# Autodesk Inventor assembly: X_Carriage_V2_1
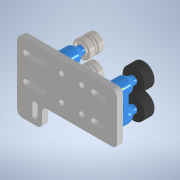
[picture p0: Inventor's stored thumbnail of the model, 180x180]
Saved by Autodesk Inventor 2021 (Build 250183000, 183)
## iProperties
Created: 2021-06-13
Part Number: X_Carriage_V2_1
Document SubType Name: Assembly
Designer: Jorian Brusind
Author: Jorian Brusind
## Documents named in this file (6)
- C:\Users\Jorian Brusind\Documents\GitHub\PersonalProjects\HyperRail\Inventor Files\X_Carriage_V2_1.iam
- C:\Users\Jorian Brusind\Documents\GitHub\PersonalProjects\HyperRail\Inventor Files\X_Carriage_Plate.ipt
- C:\Users\Jorian Brusind\Documents\GitHub\PersonalProjects\HyperRail\Inventor Files\11mm_BearingWheel.ipt
- C:\Users\Jorian Brusind\Documents\GitHub\PersonalProjects\HyperRail\Inventor Files\4mm_Roller_Spacer_extended.ipt
- C:\Users\Jorian Brusind\Documents\GitHub\PersonalProjects\HyperRail\Inventor Files\606zz_bearing.ipt
- C:\Users\Jorian Brusind\Documents\GitHub\PersonalProjects\HyperRail\Inventor Files\Bearing_Spacer.ipt
## Components (11 placed, 5 different names)
1. X_Carriage_Plate:1 — Mate:51, Mate:53, Mate:65, Angle:1, Mate:66, Angle:2
2. 11mm_BearingWheel:1 — Flush:2, Mate:56, Mate:67
3. 11mm_BearingWheel:4 — Flush:2, Mate:57
4. 4mm_Roller_Spacer_extended:1 — Mate:53, Mate:56, Mate:57, Mate:66, Angle:2, Mate:67
5. 4mm_Roller_Spacer_extended:2 — Mate:51, Mate:62, Mate:63, Mate:64, Mate:65, Angle:1
6. 606zz_bearing:1 — Mate:68, Mate:72
7. 606zz_bearing:2 — Mate:63, Mate:71
8. 606zz_bearing:3 — Mate:64, Mate:69
9. 606zz_bearing:4 — Mate:62, Mate:70
10. Bearing_Spacer:1 — Mate:69, Mate:70, Flush:4
11. Bearing_Spacer:2 — Mate:68, Mate:71, Flush:4, Mate:72
## Relationships (22: Mate 17, Flush 3, Angle 2)
- Flush:2: 11mm_BearingWheel:1 ↔ 11mm_BearingWheel:4
- Mate:51: X_Carriage_Plate:1 ↔ 4mm_Roller_Spacer_extended:2
- Mate:53: X_Carriage_Plate:1 ↔ 4mm_Roller_Spacer_extended:1
- Mate:56: 11mm_BearingWheel:1 ↔ 4mm_Roller_Spacer_extended:1
- Mate:57: 11mm_BearingWheel:4 ↔ 4mm_Roller_Spacer_extended:1
- [Mate]: 606zz_bearing:1 ↔ 606zz_bearing:2
- [Mate]: 606zz_bearing:3 ↔ 606zz_bearing:4
- [Flush]: 606zz_bearing:1 ↔ 606zz_bearing:3
- Mate:62: 4mm_Roller_Spacer_extended:2 ↔ 606zz_bearing:4
- Mate:63: 4mm_Roller_Spacer_extended:2 ↔ 606zz_bearing:2
- Mate:64: 4mm_Roller_Spacer_extended:2 ↔ 606zz_bearing:3
- Mate:65 (-12.5 mm): X_Carriage_Plate:1 ↔ 4mm_Roller_Spacer_extended:2
- Angle:1 (0 deg): X_Carriage_Plate:1 ↔ 4mm_Roller_Spacer_extended:2
- Mate:66 (-12.5 mm): X_Carriage_Plate:1 ↔ 4mm_Roller_Spacer_extended:1
- Angle:2 (0 deg): X_Carriage_Plate:1 ↔ 4mm_Roller_Spacer_extended:1
- Mate:67: 11mm_BearingWheel:1 ↔ 4mm_Roller_Spacer_extended:1
- Mate:68: 606zz_bearing:1 ↔ Bearing_Spacer:2
- Mate:69: 606zz_bearing:3 ↔ Bearing_Spacer:1
- Mate:70: 606zz_bearing:4 ↔ Bearing_Spacer:1
- Mate:71: 606zz_bearing:2 ↔ Bearing_Spacer:2
- Flush:4: Bearing_Spacer:1 ↔ Bearing_Spacer:2
- Mate:72: 606zz_bearing:1 ↔ Bearing_Spacer:2
## Named parameters: d119_d83 = 0 mm
